# Autodesk Inventor assembly: DetektorElektronik_Stage1
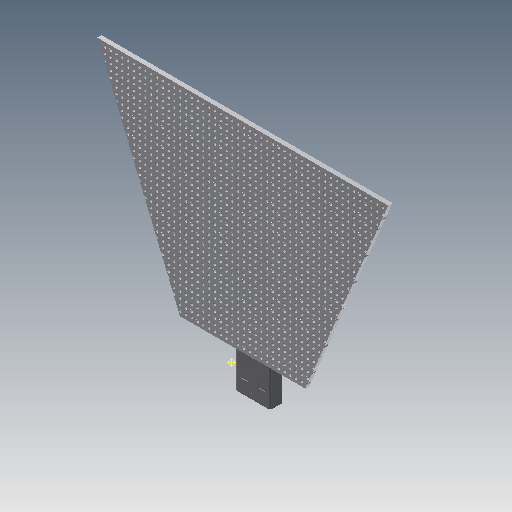
[picture p0: Inventor's stored thumbnail of the model, 512x512]
Saved by Autodesk Inventor 2018 (Build 220112000, 112)
## iProperties
Created: 2018-11-01
Part Number: DetektorElektronik_Stage1
Material: Generisch
Document SubType Name: Assembly
Designer: M.Knabel
Author: M.Knabel
## Documents named in this file (4)
- C:\Users\knabe\Documents\GitHub\COSIMA-Laserstar\CAD\Detektormodul\DetektorElektronik_Stage1.iam
- C:\Users\knabe\Documents\GitHub\COSIMA-Laserstar\CAD\Detektormodul\Detektorplatine.ipt
- C:\Users\knabe\Documents\GitHub\COSIMA-Laserstar\CAD\Detektormodul\USB_male.ipt
- C:\Users\knabe\Documents\GitHub\COSIMA-Laserstar\CAD\Oktokommander\16Bit I2C ADC+PGA - ADS1115.iam
## Components (3 placed, 3 different names)
1. Detektorplatine:1 — Fluchtend:1, Passend:1, Passend:2, Passend:3
2. USB_male:1 — Fluchtend:1, Passend:1, Passend:2
3. 16Bit I2C ADC+PGA - ADS1115:1 [sub-assembly] — Passend:3
## Relationships (4: Mate 3, Flush 1)
- Fluchtend:1 [Flush] (-16 mm): Detektorplatine:1 ↔ USB_male:1
- Passend:1 [Mate] (2 mm): Detektorplatine:1 ↔ USB_male:1
- Passend:2 [Mate] (15.647 mm): Detektorplatine:1 ↔ USB_male:1
- Passend:3 [Mate] (5 mm): Detektorplatine:1 ↔ 16Bit I2C ADC+PGA - ADS1115:1
